# Autodesk Inventor assembly: SHFL30
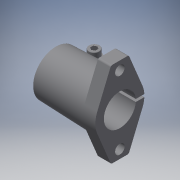
[picture p0: Inventor's stored thumbnail of the model, 180x180]
Saved by Autodesk Inventor 2019 (Build 230136000, 136)
## iProperties
Category: PARTsolutions
Company: MISUMI
Created: 2022-11-15
Part Number: SHFL30
Catalog Web Link: www.cadenas.de
Description: SHFTL, SHFML, SHFSSL, SHFL, SHFDL-Shaft Supports - Flanged Type (Precision Casting) - Long Guide Type
Vendor: MISUMI
Document SubType Name: Assembly
Designer: psAdmin
Manufacturer: MISUMI
Mass: 62.5505 g
Surface Area: 221.709 cm^2
Volume: 62.5505 cm^3
Density: 1 g/cm^3
Title: SHFL30
Author: Cadenas PARTsolutions
Comments: Shaft Supports - Flanged Type (Precision Casting) - Long Guide Type
PSOL_IDENT_0: {$CADENAS_DATA/23d-libs/misumi/metric/02_shaft_supports/shftl_asmtab.prj},200 {VTYP=3D},{STYP=ASSTAB
PSOL_IDENT_1: },{NB=SHFL30},{LINA=SHFL30},{NN=SHFTL, SHFML, SHFSSL, SHFL, SHFDL},{DATE=09.09.2019 15:26:48},{GEOMD
PSOL_IDENT_2: ATE=20.05.2016 01:01:23},{VERSION=},{LINEID=190},{WBVAR=MAT,ST},{WBNUMERIC=}  {NB=SHFL30},{LINA=SHFL
PSOL_IDENT_3: 30},{KT=DUMMY},{PN=SHFL30},{TYPE=SHFL},{MAT=514},{ST=Clear Anodize},{AC=Hexagon Socket Head Cap Scre
PSOL_IDENT_4: ws 2 Pcs. (SUS)},{D=30},{L=80},{T=60},{TT=12},{H=50.0},{A=46},{L1=64},{DD=9.0},{DD1=12},{D1=35},{TT1=
PSOL_IDENT_5: 2.0},{B=22},{C=2.5},{BB1=0},{BB2=0},{BB3=0},{HH=21.0},{G=15.0},{F=30},{M=M6},{THMD=6},{THDMIN=0.000}
PSOL_IDENT_6: ,{ST0='Clear Anodize','Clear Anodize','Black Anodize','Black Anodize'},{MASS=156},{MAT1='1045','1045
PSOL_IDENT_7: Carbon Steel','514','Aluminum Casting Alloy 514.0','304','304 Stainless Steel'},{DM=6},{HM=20.000},
PSOL_IDENT_8: {MASSS=450},{MASSA=156},{PPATH=shftl/shftl_templ.prj}
NB: SHFL30
NN: SHFTL, SHFML, SHFSSL, SHFL, SHFDL
NT: Shaft Supports - Flanged Type (Precision Casting) - Long Guide Type
NBSYN: $PN.
LINA: SHFL30
CATALOG: Misumi
PN: SHFL30
MAT: Aluminum Casting Alloy 514.0
ST: Clear Anodize
AC: Hexagon Socket Head Cap Screws 2 Pcs. (SUS)
D: 30
L: 80
T: 60
TT: 12
H: 50
A: 46
L1: 64
DD: 9
DD1: 12
D1: 35
TT1: 2
B: 22
C: 2.5
HH: 21
G: 15
F: 30
M: M6
MASS: 156
SUPPLIER: MISUMI
ARTICLENO: SHFL30
BOMINFO: SHFL30
CREATOR: CADENAS GmbH
## Documents named in this file (3)
- e:\temp\worker_COMMON_6\temp\tmp_5544_280_Kunoj\format_0\SHFL30.iam
- e:\temp\worker_COMMON_6\temp\tmp_5544_280_Kunoj\format_0\SHFTL30_b.ipt
- e:\temp\worker_COMMON_6\temp\tmp_5544_280_Kunoj\format_0\Slotted head cap screw ISO 4762 - M6x20.ipt
## Components (3 placed, 2 different names)
1. SHFTL30_b:1 — body_screw_Z@1 <-> IP1_Z@2, body_to_screw2_Z@1 <-> IP1_Z@3
2. Slotted head cap screw ISO 4762 - M6x20:1 — body_screw_Z@1 <-> IP1_Z@2
3. Slotted head cap screw ISO 4762 - M6x20:2 — body_to_screw2_Z@1 <-> IP1_Z@3
## Relationships (2: Mate 2)
- body_screw_Z@1 <-> IP1_Z@2 [Mate]: SHFTL30_b:1 ↔ Slotted head cap screw ISO 4762 - M6x20:1
- body_to_screw2_Z@1 <-> IP1_Z@3 [Mate]: SHFTL30_b:1 ↔ Slotted head cap screw ISO 4762 - M6x20:2
